# Autodesk Inventor assembly: assembly_connector
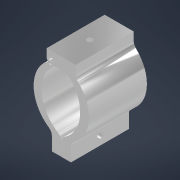
[picture p0: Inventor's stored thumbnail of the model, 180x180]
Saved by Autodesk Inventor 2021 (Build 250183000, 183)
## iProperties
Created: 2021-05-17
Part Number: assembly_connector
Document SubType Name: Assembly
Designer: chick
Mass: 1278.94 g
Surface Area: 884.205 cm^2
Volume: 473.682 cm^3
Density: 2.7 g/cm^3
Author: chick
## Documents named in this file (9)
- C:\Users\Watchdog\OneDrive - Flinders\Advn Mech Design Shared\6_Development\2_Design\inventor\connection\assembly_connector.iam
- C:\Users\Watchdog\OneDrive - Flinders\Advn Mech Design Shared\6_Development\2_Design\inventor\connection\left_part.ipt
- C:\Users\Watchdog\OneDrive - Flinders\Advn Mech Design Shared\6_Development\2_Design\inventor\connection\Hinge.ipt
- C:\Users\Watchdog\OneDrive - Flinders\Advn Mech Design Shared\6_Development\2_Design\inventor\connection\assembly_connector\AIP\FEA\dm8i2qu8w.fins
- C:\Users\Watchdog\OneDrive - Flinders\Advn Mech Design Shared\6_Development\2_Design\inventor\connection\assembly_connector\AIP\FEA\dm8i2qu8w.fsat
- C:\Users\Watchdog\OneDrive - Flinders\Advn Mech Design Shared\6_Development\2_Design\inventor\connection\assembly_connector\AIP\FEA\dm8i2qu8w.ftes
- C:\Users\Watchdog\OneDrive - Flinders\Advn Mech Design Shared\6_Development\2_Design\inventor\connection\assembly_connector\AIP\FEA\dm8i2qu8w.fwiz
- C:\Users\Watchdog\OneDrive - Flinders\Advn Mech Design Shared\6_Development\2_Design\inventor\connection\assembly_connector\AIP\FEA\dm8i2qu9s.fmsh
- C:\Users\Watchdog\OneDrive - Flinders\Advn Mech Design Shared\6_Development\2_Design\inventor\connection\assembly_connector\AIP\FEA\dm8i2qu9t.fres
## Components (2 placed, 2 different names)
1. left_part:1 — Mate:2, Mate:3, Flush:2
2. Hinge:1 — Mate:2, Mate:3
## Relationships (3: Mate 2, Flush 1)
- Mate:2: left_part:1 ↔ Hinge:1
- Mate:3: left_part:1 ↔ Hinge:1
- Flush:2 (50 mm): left_part:1
## Named parameters: sa_0 = 3.403e-10, sa_1 = -41202, sa_2 = 41202
note: some values were not read from the file. Shown as the stored number, unit unknown: "sa_0", "sa_1", "sa_2".
